# Autodesk Inventor assembly: Zusammenbau_V2
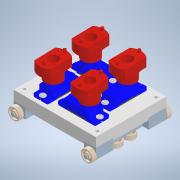
[picture p0: Inventor's stored thumbnail of the model, 180x180]
Saved by Autodesk Inventor 2022 (Build 260153000, 153)
## iProperties
Created: 2022-04-26
Part Number: Zusammenbau_V2
Document SubType Name: Assembly
Designer: 123St
Author: 123St
## Documents named in this file (7)
- D:\Eigene Dateien\Desktop\UNI\Semester 5\Praktikum\DaVinci\Ueberarbeiteter DaVincikopf\Zusammenbau_V2.iam
- D:\Eigene Dateien\Desktop\UNI\Semester 5\Praktikum\DaVinci\Ueberarbeiteter DaVincikopf\Fuehrungsgrundplatte_V2.ipt
- D:\Eigene Dateien\Desktop\UNI\Semester 5\Praktikum\DaVinci\Ueberarbeiteter DaVincikopf\sg90-micro-servo-9g-tower-pro-1.snapshot.3\SG90 - Micro Servo 9g - Tower Pro.iam
- D:\Eigene Dateien\Desktop\UNI\Semester 5\Praktikum\DaVinci\Ueberarbeiteter DaVincikopf\Fuehrungslagerhalter_v2.ipt
- D:\Eigene Dateien\Desktop\UNI\Semester 5\Praktikum\DaVinci\Ueberarbeiteter DaVincikopf\126017015-9-bb-623-a500-70-es\bb-623-a500-70-es.iam
- D:\Eigene Dateien\Desktop\UNI\Semester 5\Praktikum\DaVinci\Ueberarbeiteter DaVincikopf\Adaptation_on_OPdevside_4_1.ipt
- D:\Eigene Dateien\Desktop\UNI\Semester 5\Praktikum\DaVinci\Ueberarbeiteter DaVincikopf\SG90 - Micro Servo 9g - Tower Pro.6_BS EN ISO 7045 - M2 x 4 - Z - 4S.ipt
## Components (23 placed, 6 different names)
1. Fuehrungsgrundplatte_V2:1 — Passend:3, Passend:4, Passend:5, Passend:6, Passend:7, Passend:8, Passend:9, Passend:10, Passend:11, Passend:12, Passend:13, Passend:14, Passend:15, Passend:16, Passend:17, Passend:18, Passend:19, Passend:20
2. SG90 - Micro Servo 9g - Tower Pro:1 [sub-assembly] — Passend:9, Passend:10, Passend:11, Drehbar:10
3. SG90 - Micro Servo 9g - Tower Pro:2 [sub-assembly] — Passend:12, Passend:13, Passend:14, Drehbar:12
4. SG90 - Micro Servo 9g - Tower Pro:3 [sub-assembly] — Passend:4, Passend:5, Passend:6, Drehbar:11
5. SG90 - Micro Servo 9g - Tower Pro:4 [sub-assembly] — Passend:3, Passend:7, Passend:8, Drehbar:9
6. Fuehrungslagerhalter_v2:1 — Passend:15, Passend:16, Passend:17, Drehbar:1, Drehbar:2, Drehbar:6, Drehbar:8
7. Fuehrungslagerhalter_v2:2 — Passend:18, Passend:19, Passend:20, Drehbar:3, Drehbar:4, Drehbar:5, Drehbar:7
8. bb-623-a500-70-es:1 [sub-assembly] — Drehbar:6
9. bb-623-a500-70-es:2 [sub-assembly] — Drehbar:5
10. bb-623-a500-70-es:3 [sub-assembly] — Drehbar:8
11. bb-623-a500-70-es:4 [sub-assembly] — Drehbar:7
12. bb-623-a500-70-es:5 [sub-assembly] — Drehbar:1
13. bb-623-a500-70-es:6 [sub-assembly] — Drehbar:2
14. bb-623-a500-70-es:7 [sub-assembly] — Drehbar:3
15. bb-623-a500-70-es:8 [sub-assembly] — Drehbar:4
16. Adaptation_on_OPdevside_4_1:1 — Drehbar:9, Drehbar:13
17. Adaptation_on_OPdevside_4_1:2 — Drehbar:12, Drehbar:16
18. Adaptation_on_OPdevside_4_1:3 — Drehbar:11, Drehbar:14
19. Adaptation_on_OPdevside_4_1:4 — Drehbar:10, Drehbar:15
20. SG90 - Micro Servo 9g - Tower Pro.6_BS EN ISO 7045 - M2 x 4 - Z - 4S:1 — Drehbar:16
21. SG90 - Micro Servo 9g - Tower Pro.6_BS EN ISO 7045 - M2 x 4 - Z - 4S:2 — Drehbar:14
22. SG90 - Micro Servo 9g - Tower Pro.6_BS EN ISO 7045 - M2 x 4 - Z - 4S:3 — Drehbar:15
23. SG90 - Micro Servo 9g - Tower Pro.6_BS EN ISO 7045 - M2 x 4 - Z - 4S:4 — Drehbar:13
## Relationships (34: Mate 18, RevoluteJoint 16)
- Passend:3 [Mate]: Fuehrungsgrundplatte_V2:1 ↔ SG90 - Micro Servo 9g - Tower Pro:4
- Passend:4 [Mate]: Fuehrungsgrundplatte_V2:1 ↔ SG90 - Micro Servo 9g - Tower Pro:3
- Passend:5 [Mate]: Fuehrungsgrundplatte_V2:1 ↔ SG90 - Micro Servo 9g - Tower Pro:3
- Passend:6 [Mate]: Fuehrungsgrundplatte_V2:1 ↔ SG90 - Micro Servo 9g - Tower Pro:3
- Passend:7 [Mate]: Fuehrungsgrundplatte_V2:1 ↔ SG90 - Micro Servo 9g - Tower Pro:4
- Passend:8 [Mate]: Fuehrungsgrundplatte_V2:1 ↔ SG90 - Micro Servo 9g - Tower Pro:4
- Passend:9 [Mate]: Fuehrungsgrundplatte_V2:1 ↔ SG90 - Micro Servo 9g - Tower Pro:1
- Passend:10 [Mate]: Fuehrungsgrundplatte_V2:1 ↔ SG90 - Micro Servo 9g - Tower Pro:1
- Passend:11 [Mate]: Fuehrungsgrundplatte_V2:1 ↔ SG90 - Micro Servo 9g - Tower Pro:1
- Passend:12 [Mate]: Fuehrungsgrundplatte_V2:1 ↔ SG90 - Micro Servo 9g - Tower Pro:2
- Passend:13 [Mate]: Fuehrungsgrundplatte_V2:1 ↔ SG90 - Micro Servo 9g - Tower Pro:2
- Passend:14 [Mate]: Fuehrungsgrundplatte_V2:1 ↔ SG90 - Micro Servo 9g - Tower Pro:2
- Passend:15 [Mate]: Fuehrungsgrundplatte_V2:1 ↔ Fuehrungslagerhalter_v2:1
- Passend:16 [Mate]: Fuehrungsgrundplatte_V2:1 ↔ Fuehrungslagerhalter_v2:1
- Passend:17 [Mate]: Fuehrungsgrundplatte_V2:1 ↔ Fuehrungslagerhalter_v2:1
- Passend:18 [Mate]: Fuehrungsgrundplatte_V2:1 ↔ Fuehrungslagerhalter_v2:2
- Passend:19 [Mate]: Fuehrungsgrundplatte_V2:1 ↔ Fuehrungslagerhalter_v2:2
- Passend:20 [Mate]: Fuehrungsgrundplatte_V2:1 ↔ Fuehrungslagerhalter_v2:2
- Drehbar:1 [RevoluteJoint]: Fuehrungslagerhalter_v2:1 ↔ bb-623-a500-70-es:5
- Drehbar:2 [RevoluteJoint]: Fuehrungslagerhalter_v2:1 ↔ bb-623-a500-70-es:6
- Drehbar:3 [RevoluteJoint]: Fuehrungslagerhalter_v2:2 ↔ bb-623-a500-70-es:7
- Drehbar:4 [RevoluteJoint]: Fuehrungslagerhalter_v2:2 ↔ bb-623-a500-70-es:8
- Drehbar:5 [RevoluteJoint]: Fuehrungslagerhalter_v2:2 ↔ bb-623-a500-70-es:2
- Drehbar:6 [RevoluteJoint]: Fuehrungslagerhalter_v2:1 ↔ bb-623-a500-70-es:1
- Drehbar:7 [RevoluteJoint]: Fuehrungslagerhalter_v2:2 ↔ bb-623-a500-70-es:4
- Drehbar:8 [RevoluteJoint]: Fuehrungslagerhalter_v2:1 ↔ bb-623-a500-70-es:3
- Drehbar:9 [RevoluteJoint]: SG90 - Micro Servo 9g - Tower Pro:4 ↔ Adaptation_on_OPdevside_4_1:1
- Drehbar:10 [RevoluteJoint]: SG90 - Micro Servo 9g - Tower Pro:1 ↔ Adaptation_on_OPdevside_4_1:4
- Drehbar:11 [RevoluteJoint]: SG90 - Micro Servo 9g - Tower Pro:3 ↔ Adaptation_on_OPdevside_4_1:3
- Drehbar:12 [RevoluteJoint]: SG90 - Micro Servo 9g - Tower Pro:2 ↔ Adaptation_on_OPdevside_4_1:2
- Drehbar:13 [RevoluteJoint]: Adaptation_on_OPdevside_4_1:1 ↔ SG90 - Micro Servo 9g - Tower Pro.6_BS EN ISO 7045 - M2 x 4 - Z - 4S:4
- Drehbar:14 [RevoluteJoint]: Adaptation_on_OPdevside_4_1:3 ↔ SG90 - Micro Servo 9g - Tower Pro.6_BS EN ISO 7045 - M2 x 4 - Z - 4S:2
- Drehbar:15 [RevoluteJoint]: Adaptation_on_OPdevside_4_1:4 ↔ SG90 - Micro Servo 9g - Tower Pro.6_BS EN ISO 7045 - M2 x 4 - Z - 4S:3
- Drehbar:16 [RevoluteJoint]: Adaptation_on_OPdevside_4_1:2 ↔ SG90 - Micro Servo 9g - Tower Pro.6_BS EN ISO 7045 - M2 x 4 - Z - 4S:1
